# Autodesk Inventor assembly: писюны
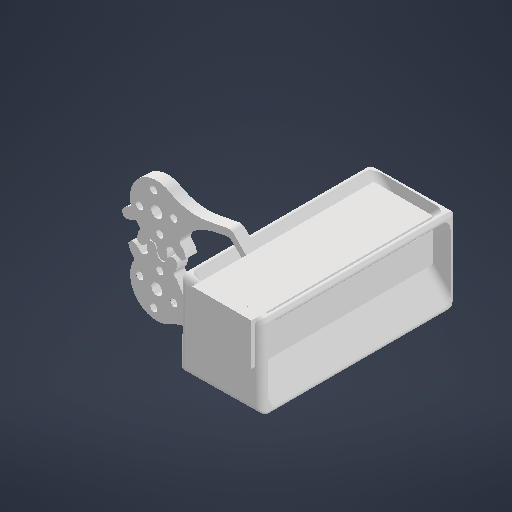
[picture p0: Inventor's stored thumbnail of the model, 512x512]
Saved by Autodesk Inventor 2025 (Build 290162000, 162)
## iProperties
Created: 2024-12-28
Part Number: писюны
Document SubType Name: Assembly
Designer: Phantom
Author: Phantom
## Documents named in this file (4)
- C:\Users\GameHD\Desktop\phantom 16950\писюны.iam
- C:\Users\GameHD\Desktop\phantom 16950\am-5401 Sample.ipt
- C:\Users\GameHD\Desktop\phantom 16950\писюн.ipt
- C:\Users\GameHD\Desktop\phantom 16950\писюн 2.ipt
## Components (3 placed, 3 different names)
1. писюн:1 — Совмещение:1, Заподлицо:1, Совмещение:3
2. писюн 2:1 — Совмещение:1, Совмещение:2, Заподлицо:1, Совмещение:3
3. am-5401 Sample:1 — Совмещение:2
## Relationships (4: Mate 3, Flush 1)
- Совмещение:1 [Mate] (30 mm): писюн:1 ↔ писюн 2:1
- Совмещение:2 [Mate] (20 mm): писюн 2:1 ↔ am-5401 Sample:1
- Заподлицо:1 [Flush]: писюн:1 ↔ писюн 2:1
- Совмещение:3 [Mate]: писюн:1 ↔ писюн 2:1
